# Autodesk Inventor assembly: Denzel4500Motor
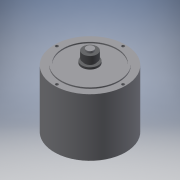
[picture p0: Inventor's stored thumbnail of the model, 180x180]
Saved by Autodesk Inventor 2018 (Build 220112000, 112)
## iProperties
Created: 2018-10-10
Part Number: Denzel4500Motor
Document SubType Name: Assembly
Designer: eroldan
Author: eroldan
## Documents named in this file (3)
- C:\Users\eroldan\Desktop\3dprojects\OpenEmoto\OtherParts\Denzel4500Motor.iam
- C:\Users\eroldan\Desktop\3dprojects\OpenEmoto\OtherParts\Denzel4500Motor.ipt
- C:\Users\eroldan\Desktop\3dprojects\OpenEmoto\OtherParts\DriveSprocket12T.ipt
## Components (2 placed, 2 different names)
1. Denzel4500Motor:1 — Mate:1, Flush:1
2. DriveSprocket12T:1 — Mate:1, Flush:1
## Relationships (2: Mate 1, Flush 1)
- Mate:1: Denzel4500Motor:1 ↔ DriveSprocket12T:1
- Flush:1 (-8 mm): Denzel4500Motor:1 ↔ DriveSprocket12T:1
